# Autodesk Inventor assembly: motor_assembly
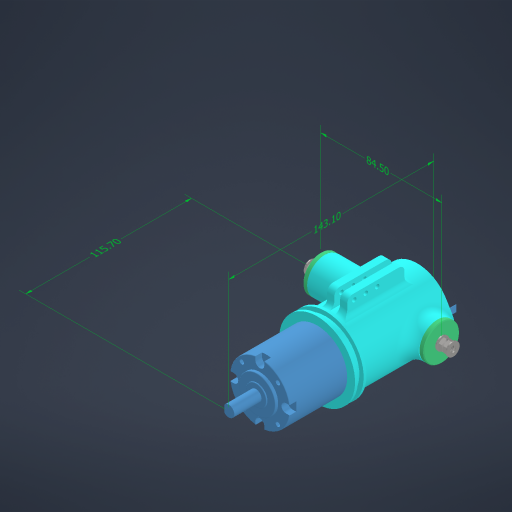
[picture p0: Inventor's stored thumbnail of the model, 512x512]
Saved by Autodesk Inventor 2024 (Build 280153000, 153)
## iProperties
Created: 2023-04-15
Part Number: motor_assembly
Document SubType Name: Assembly
Designer: user
Author: user
## Documents named in this file (7)
- D:\Docs\Robot\3d\motor_assembly\side_left\motor_assembly_M.iam
- D:\Docs\Robot\3d\default_components\motor.ipt
- D:\Docs\Robot\3d\motor_assembly\side_left\lower_arm.ipt
- D:\Docs\Robot\3d\motor_assembly\side_left\bushing.ipt
- D:\Docs\Robot\3d\motor_assembly\604zz_bearing.ipt
- C:\Users\user\Documents\Inventor\Content Center Files\R2024\ru-RU\DIN 934\DIN 934 - M4 x 0,7.ipt
- C:\Users\user\Documents\Inventor\Content Center Files\R2024\ru-RU\DIN 125-1  A\DIN 125 - A 4,3.ipt
## Components (14 placed, 6 different names)
1. motor:1 — Совмещение:1, Совмещение:2, Совмещение:3, Заподлицо:1
2. lower_arm:1 — Заподлицо:1, Заподлицо:2, Заподлицо:3, Совмещение:4, С поворотом:1
3. bushing:1 — Заподлицо:2, Заподлицо:3, Угол:1, Вставка:2, Вставка:3
4. bushing:2 — С поворотом:1, Угол:2, Вставка:1, Вставка:7
5. 604zz_bearing:1 — Вставка:1
6. 604zz_bearing:2 — Вставка:2
7. DIN 934 - заменено на DIN EN 24032/28673/28674 M4:1 — Вставка:4, Вставка:5
8. DIN 934 - заменено на DIN EN 24032/28673/28674 M4:2 — Вставка:5, Вставка:6
9. DIN 934 - заменено на DIN EN 24032/28673/28674 M4:3 — Вставка:8, Вставка:9
10. DIN 934 - заменено на DIN EN 24032/28673/28674 M4:4 — Вставка:9, Вставка:10
11. DIN 125-1 A A 4,3:1 — Вставка:3, Вставка:4
12. DIN 125-1 A A 4,3:2 — Вставка:6
13. DIN 125-1 A A 4,3:3 — Вставка:7, Вставка:8
14. DIN 125-1 A A 4,3:4 — Вставка:10
## Relationships (20: Insert 10, Mate 4, Flush 3, Angle 2, RevoluteJoint 1)
- Совмещение:1 [Mate]: motor:1
- Совмещение:2 [Mate]: motor:1
- Совмещение:3 [Mate]: motor:1
- Заподлицо:1 [Flush]: motor:1 ↔ lower_arm:1
- Заподлицо:2 [Flush]: lower_arm:1 ↔ bushing:1
- Заподлицо:3 [Flush]: lower_arm:1 ↔ bushing:1
- Совмещение:4 [Mate]: lower_arm:1
- Угол:1 [Angle] (0 deg): bushing:1
- С поворотом:1 [RevoluteJoint]: lower_arm:1 ↔ bushing:2
- Угол:2 [Angle] (0 deg): bushing:2
- Вставка:1 [Insert]: bushing:2 ↔ 604zz_bearing:1
- Вставка:2 [Insert]: bushing:1 ↔ 604zz_bearing:2
- Вставка:3 [Insert]: bushing:1 ↔ DIN 125-1 A A 4,3:1
- Вставка:4 [Insert]: DIN 934 - заменено на DIN EN 24032/28673/28674 M4:1 ↔ DIN 125-1 A A 4,3:1
- Вставка:5 [Insert]: DIN 934 - заменено на DIN EN 24032/28673/28674 M4:1 ↔ DIN 934 - заменено на DIN EN 24032/28673/28674 M4:2
- Вставка:6 [Insert]: DIN 934 - заменено на DIN EN 24032/28673/28674 M4:2 ↔ DIN 125-1 A A 4,3:2
- Вставка:7 [Insert]: bushing:2 ↔ DIN 125-1 A A 4,3:3
- Вставка:8 [Insert]: DIN 934 - заменено на DIN EN 24032/28673/28674 M4:3 ↔ DIN 125-1 A A 4,3:3
- Вставка:9 [Insert]: DIN 934 - заменено на DIN EN 24032/28673/28674 M4:3 ↔ DIN 934 - заменено на DIN EN 24032/28673/28674 M4:4
- Вставка:10 [Insert]: DIN 934 - заменено на DIN EN 24032/28673/28674 M4:4 ↔ DIN 125-1 A A 4,3:4
